# Autodesk Inventor assembly: Leg
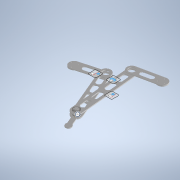
[picture p0: Inventor's stored thumbnail of the model, 180x180]
Saved by Autodesk Inventor 2022 (Build 260153000, 153)
## iProperties
Created: 2022-03-17
Part Number: Leg
Document SubType Name: Assembly
Designer: br4ch
Author: br4ch
## Documents named in this file (8)
- C:\Users\br4ch\M-and-Ms\Strirus\Leg.iam
- C:\Users\br4ch\M-and-Ms\Strirus\psmall.ipt
- C:\Users\br4ch\M-and-Ms\Strirus\p2.ipt
- C:\Users\br4ch\M-and-Ms\Strirus\p1.ipt
- C:\Users\br4ch\M-and-Ms\Strirus\Leg\Design Accelerator\Bearing2.iam
- C:\Users\br4ch\M-and-Ms\Strirus\cork.ipt
- C:\Users\br4ch\M-and-Ms\Strirus\Shaft1.ipt
- C:\Users\br4ch\M-and-Ms\Strirus\Leg\Design Accelerator\Bearing3.iam
## Components (9 placed, 6 different names)
1. psmall:1 — Mate:6, Cylindrical:6
2. psmall:2 — Flush:8, Cylindrical:7
3. p2:1 — Flush:5, Cylindrical:3, Flush:8, Cylindrical:7
4. p1:1 — Mate:1, Flush:1, Mate:6, Cylindrical:6
5. Bearing:1 [sub-assembly] — Mate:1, Flush:1, Cylindrical:1, Mate:2
6. cork:1 — Cylindrical:1, Mate:2, Cylindrical:2, Mate:3
7. Shaft:2 — Cylindrical:2, Mate:3, Cylindrical:4, Mate:4
8. Bearing:2 [sub-assembly] — Flush:5, Cylindrical:3, Cylindrical:4, Mate:4, Cylindrical:5, Mate:5
9. cork:2 — Cylindrical:5, Mate:5
## Relationships (16: CylindricalJoint 7, Mate 6, Flush 3)
- Mate:1: p1:1 ↔ Bearing:1
- Flush:1: p1:1 ↔ Bearing:1
- Cylindrical:1: Bearing:1 ↔ cork:1
- Mate:2: Bearing:1 ↔ cork:1
- Cylindrical:2: cork:1 ↔ Shaft:2
- Mate:3: cork:1 ↔ Shaft:2
- Flush:5: p2:1 ↔ Bearing:2
- Cylindrical:3: p2:1 ↔ Bearing:2
- Cylindrical:4: Shaft:2 ↔ Bearing:2
- Mate:4: Shaft:2 ↔ Bearing:2
- Cylindrical:5: Bearing:2 ↔ cork:2
- Mate:5: Bearing:2 ↔ cork:2
- Mate:6 (5 mm): psmall:1 ↔ p1:1
- Cylindrical:6: psmall:1 ↔ p1:1
- Flush:8 (5 mm): psmall:2 ↔ p2:1
- Cylindrical:7: psmall:2 ↔ p2:1
